# Autodesk Inventor assembly: LargeCBackingPoly
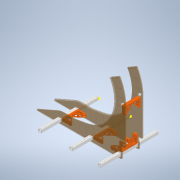
[picture p0: Inventor's stored thumbnail of the model, 180x180]
Saved by Autodesk Inventor 2020 (Build 240168000, 168)
## iProperties
Created: 2020-01-20
Part Number: LargeCBackingPoly
Document SubType Name: Assembly
Designer: srini
Author: srini
## Documents named in this file (5)
- C:\Users\srini\Documents\FRC\2020\IntakeShooter\LargeCBackingPoly.iam
- C:\Users\srini\Documents\FRC\2020\IntakeShooter\OutsideCLarge.ipt
- C:\Users\srini\Documents\FRC\2020\IntakeShooter\OutsideCSmall.ipt
- C:\Users\srini\Documents\FRC\2020\IntakeShooter\IndexerSpacer5_5_2.ipt
- C:\Users\srini\Documents\FRC\2020\IntakeShooter\1x1x20.25.ipt
## Components (12 placed, 4 different names)
1. OutsideCLarge:1 — Insert:1, Insert:2
2. OutsideCSmall:1 — Insert:1, Insert:2, Insert:3, Insert:4, Insert:5, Insert:6, Insert:7, Insert:8, Insert:9, Insert:10, Insert:11, Insert:12
3. IndexerSpacer5_5_2:1 — Insert:5, Insert:6, Insert:18, Insert:20
4. IndexerSpacer5_5_2:2 — Insert:9, Insert:10
5. IndexerSpacer5_5_2:3 — Insert:7, Insert:8, Insert:21, Insert:22
6. IndexerSpacer5_5_2:4 — Insert:11, Insert:12, Insert:14
7. IndexerSpacer5_5_2:5 — Insert:3, Insert:4, Insert:13, Insert:17, Insert:19
8. OutsideCSmall:2 — Insert:13, Insert:14, Insert:15, Insert:16
9. OutsideCLarge:2 — Insert:15, Insert:16
10. 1x1x20.25:1 — Insert:17, Insert:19
11. 1x1x20.25:2 — Insert:18, Insert:20
12. 1x1x20.25:3 — Insert:21, Insert:22
## Relationships (22: Insert 22)
- Insert:1: OutsideCLarge:1 ↔ OutsideCSmall:1
- Insert:2: OutsideCLarge:1 ↔ OutsideCSmall:1
- Insert:3: OutsideCSmall:1 ↔ IndexerSpacer5_5_2:5
- Insert:4: OutsideCSmall:1 ↔ IndexerSpacer5_5_2:5
- Insert:5: OutsideCSmall:1 ↔ IndexerSpacer5_5_2:1
- Insert:6: OutsideCSmall:1 ↔ IndexerSpacer5_5_2:1
- Insert:7: OutsideCSmall:1 ↔ IndexerSpacer5_5_2:3
- Insert:8: OutsideCSmall:1 ↔ IndexerSpacer5_5_2:3
- Insert:9: OutsideCSmall:1 ↔ IndexerSpacer5_5_2:2
- Insert:10: OutsideCSmall:1 ↔ IndexerSpacer5_5_2:2
- Insert:11: OutsideCSmall:1 ↔ IndexerSpacer5_5_2:4
- Insert:12: OutsideCSmall:1 ↔ IndexerSpacer5_5_2:4
- Insert:13: IndexerSpacer5_5_2:5 ↔ OutsideCSmall:2
- Insert:14: IndexerSpacer5_5_2:4 ↔ OutsideCSmall:2
- Insert:15: OutsideCSmall:2 ↔ OutsideCLarge:2
- Insert:16: OutsideCSmall:2 ↔ OutsideCLarge:2
- Insert:17: IndexerSpacer5_5_2:5 ↔ 1x1x20.25:1
- Insert:18: IndexerSpacer5_5_2:1 ↔ 1x1x20.25:2
- Insert:19: IndexerSpacer5_5_2:5 ↔ 1x1x20.25:1
- Insert:20: IndexerSpacer5_5_2:1 ↔ 1x1x20.25:2
- Insert:21: IndexerSpacer5_5_2:3 ↔ 1x1x20.25:3
- Insert:22: IndexerSpacer5_5_2:3 ↔ 1x1x20.25:3
